# Autodesk Inventor assembly: Baugruppe4
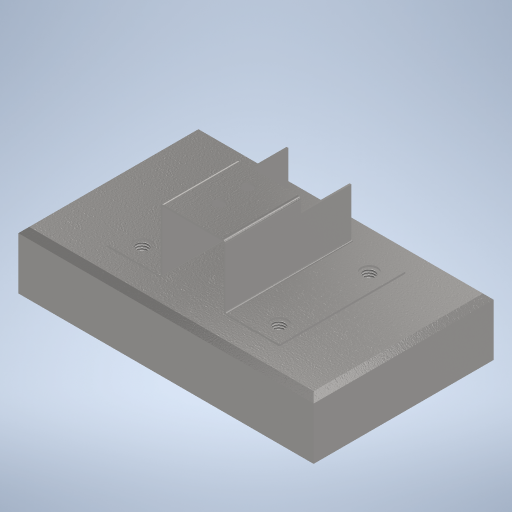
[picture p0: Inventor's stored thumbnail of the model, 512x512]
Saved by Autodesk Inventor 2024 (Build 280153000, 153)
## iProperties
Created: 2024-01-16
Part Number: Baugruppe4
Document SubType Name: Assembly
Designer: ffogue
Author: ffogue
## Documents named in this file (3)
- C:\Users\ffogue\OneDrive - MuM - OM\Dokumente\Inventor\Motor\Baugruppe4.iam
- C:\Users\ffogue\OneDrive - MuM - OM\Dokumente\Inventor\Motor\Grundplatte.ipt
- C:\Users\ffogue\OneDrive - MuM - OM\Dokumente\Inventor\Motor\Bügelbefestigung.ipt
## Components (2 placed, 2 different names)
1. Grundplatte:1 — Einfügen:1
2. Bügelbefestigung:1 — Einfügen:1
## Relationships (1: Insert 1)
- Einfügen:1 [Insert]: Grundplatte:1 ↔ Bügelbefestigung:1
